# Autodesk Inventor assembly: Gearbox
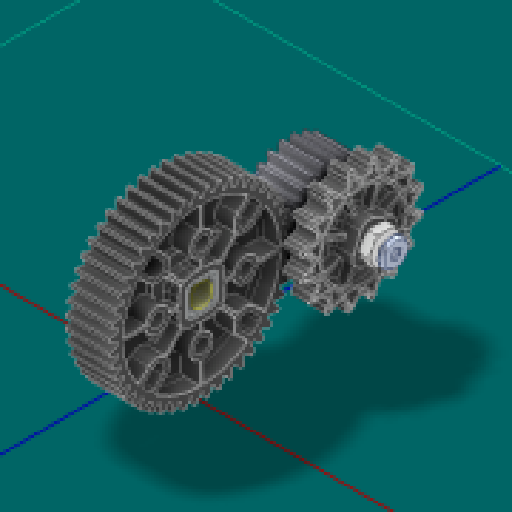
[picture p0: Inventor's stored thumbnail of the model, 512x512]
Saved by Autodesk Inventor 2025 (Build 290162000, 162)
## iProperties
Created: 2024-10-21
Part Number: Gearbox
Document SubType Name: Assembly
Designer: averey
Author: averey
## Documents named in this file (15)
- C:\Users\avere\VEX\High Stakes\CAD\V2\Intake\Gearbox.iam
- Gearbox Left.iam
- C:\Users\avere\VEX\High Stakes\CAD\ROBOPROS-CAD-Inventor\Motion\Gears\HS Gear\HS 24T Gear, No Insert.iam
- C:\Users\avere\VEX\High Stakes\CAD\ROBOPROS-CAD-Inventor\Motion\Sprockets\6P Sprocket\6P 16T Sprocket, No Insert.iam
- C:\Users\avere\VEX\High Stakes\CAD\V2\Intake\Custom Parts\Gearbox Gusset.ipt
- C:\Users\avere\VEX\High Stakes\CAD\ROBOPROS-CAD-Inventor\Motion\Gears\HS Gear\HS 48T Gear, No Insert.iam
- C:\Users\avere\VEX\High Stakes\CAD\ROBOPROS-CAD-Inventor\Motion\Gears\HS Gear.iam
- C:\Users\avere\VEX\High Stakes\CAD\ROBOPROS-CAD-Inventor\Structure\Hardware\Nut Nylon\Nut Nylon - White.ipt
- C:\Users\avere\VEX\High Stakes\CAD\ROBOPROS-CAD-Inventor\Structure\Hardware\Nut Nylon.ipt
- C:\Users\avere\VEX\High Stakes\CAD\ROBOPROS-CAD-Inventor\Structure\Hardware\Nut Thin Nylock.ipt
- C:\Users\avere\VEX\High Stakes\CAD\ROBOPROS-CAD-Inventor\Structure\Hardware\Screw Steel - Star\SScrew Star Smooth 1.500.ipt
- C:\Users\avere\VEX\High Stakes\CAD\ROBOPROS-CAD-Inventor\Structure\Hardware\Screw Steel - Star.ipt
- C:\Users\avere\VEX\High Stakes\CAD\ROBOPROS-CAD-Inventor\Motion\Shaft HS\HS Spacer\HSpacer .0625.ipt
- C:\Users\avere\VEX\High Stakes\CAD\ROBOPROS-CAD-Inventor\Motion\Shaft HS\HS Spacer.ipt
- C:\Users\avere\VEX\High Stakes\CAD\ROBOPROS-CAD-Inventor\Motion\Sprockets\6P Sprocket.iam
## Components (8 placed, 8 different names)
1. HS 24T Gear, No Insert:1 [sub-assembly] — Insert:3
2. 6P 16T Sprocket, No Insert:1 [sub-assembly] — Insert:4
3. Gearbox Gusset:1 — Mate:2, Mate:3, Insert:3, Mate:4, Insert:5, Insert:7
4. HS 48T Gear, No Insert:2 [sub-assembly]
5. Nut Nylon - White:1 — Insert:4, Insert:6
6. Nut Thin Nylock:1 — Insert:5
7. SScrew Star Smooth 1.500:1 — Insert:6
8. HSpacer .0625:1 — Insert:7
## Relationships (11: Insert 7, Mate 4)
- [Insert]: HS 24T Gear, No Insert:1 ↔ 6P 16T Sprocket, No Insert:1
- [Mate]: HS 24T Gear, No Insert:1 ↔ Gearbox Gusset:1
- [Insert] (1.5875 mm): Gearbox Gusset:1 ↔ HS 48T Gear, No Insert:2
- Mate:2: Gearbox Gusset:1
- Mate:3: Gearbox Gusset:1
- Insert:3 (0.5969 mm): HS 24T Gear, No Insert:1 ↔ Gearbox Gusset:1
- Mate:4: Gearbox Gusset:1
- Insert:4: 6P 16T Sprocket, No Insert:1 ↔ Nut Nylon - White:1
- Insert:5: Gearbox Gusset:1 ↔ Nut Thin Nylock:1
- Insert:6 (1.5875 mm): Nut Nylon - White:1 ↔ SScrew Star Smooth 1.500:1
- Insert:7: Gearbox Gusset:1 ↔ HSpacer .0625:1
